# Autodesk Inventor assembly: 8059120 SDBT-MSX-1L-PU-E-0.3-N-M8
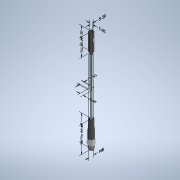
[picture p0: Inventor's stored thumbnail of the model, 180x180]
Saved by Autodesk Inventor 2021 (Build 250183000, 183)
## iProperties
Category: PARTsolutions
Company: FESTO
Created: 2025-06-25
Part Number: 8059120 SDBT-MSX-1L-PU-E-0.3-N-M8
Catalog Web Link: www.cadenas.de
Description: SDBT-MSX-proximity sensor
Vendor: FESTO
Document SubType Name: Assembly
Designer: psAdmin
Manufacturer: FESTO
Mass: 10 g
Surface Area: 28.8721 cm^2
Volume: 3.2173 cm^3
Density: 3.1082 g/cm^3
Title: 8059120 SDBT-MSX-1L-PU-E-0.3-N-M8
Author: Cadenas PARTsolutions
Comments: proximity sensor
PSOL_IDENT_0: {ATYP=ASSISTANT},{DATA=script=$CADENAS_DATA/23d-libs/festo/webfesto.vbb&M_FAMILY=SDBT&M_GROUP=01&M_P
PSOL_IDENT_1: ARTNO=8059120&IDCODE1=SDBT-MSX-1L-PU-E-0.3-N-M8&IDCODE2=&customer_number_cns=&MATES=1&LOD=HI&LOCKERP=
PSOL_IDENT_2: 0&SINGLEPART=1}
NB: 8059120 SDBT-MSX-1L-PU-E-0.3-N-M8
NN: SDBT-MSX
NT: proximity sensor
NBSYN: $TNR. $TYP.
LINA: 8059120 SDBT-MSX-1L-PU-E-0.3-N-M8
CATALOG: Festo
TNR: 8059120
TYP: SDBT-MSX-1L-PU-E-0.3-N-M8
SSZ: MSX
BSA: 1L
SAD: PU
LEI: E
LL: 0.3
LEIT: N
ELA: M8
CNSMASSEXACT: 0.01
MOM: 0.1 - 0.6
GTIN: 4052568300449
REACH: Yes
REACHSVHC: Yes
REACHHAZSUBS: 7439-92-1
REACHVALDATE: 05.03.2025
SUPPLIER: FESTO
ARTICLENO: 8059120 SDBT-MSX-1L-PU-E-0.3-N-M8
BOMINFO: 8059120 SDBT-MSX-1L-PU-E-0.3-N-M8
CREATOR: CADENAS GmbH
## Documents named in this file (3)
- e:\temp\worker_COMMON_496\temp\tmp_8500_126_KNTZX\format_0\8059120 SDBT-MSX-1L-PU-E-0_3-N-M8.iam
- e:\temp\worker_COMMON_496\temp\tmp_8500_126_KNTZX\format_0\8082090 SDBT-MSX-1L-PU-E-0_3-N-M8---(part).ipt
- e:\temp\worker_COMMON_496\temp\tmp_8500_126_KNTZX\format_0\8082090 SDBT-M8---(stecker).ipt
## Components (2 placed, 2 different names)
1. 8082090 SDBT-MSX-1L-PU-E-0_3-N-M8---(part):1 — IP_XY@1 <-> ANBAU_XY@2, IP_Z@1 <-> ANBAU_Z@2, IP_YZ@1 <-> ANBAU_YZ@2
2. 8082090 SDBT-M8---(stecker):1 — IP_XY@1 <-> ANBAU_XY@2, IP_Z@1 <-> ANBAU_Z@2, IP_YZ@1 <-> ANBAU_YZ@2
## Relationships (3: Mate 2, Angle 1)
- IP_XY@1 <-> ANBAU_XY@2 [Mate]: 8082090 SDBT-MSX-1L-PU-E-0_3-N-M8---(part):1 ↔ 8082090 SDBT-M8---(stecker):1
- IP_Z@1 <-> ANBAU_Z@2 [Mate]: 8082090 SDBT-MSX-1L-PU-E-0_3-N-M8---(part):1 ↔ 8082090 SDBT-M8---(stecker):1
- IP_YZ@1 <-> ANBAU_YZ@2 [Angle] (0 deg): 8082090 SDBT-MSX-1L-PU-E-0_3-N-M8---(part):1 ↔ 8082090 SDBT-M8---(stecker):1
